# Autodesk Inventor assembly: Bracket Assembly MK6
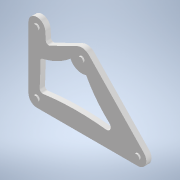
[picture p0: Inventor's stored thumbnail of the model, 180x180]
Saved by Autodesk Inventor 2021 (Build 250183000, 183)
## iProperties
Created: 2021-05-12
Part Number: Bracket Assembly MK6
Document SubType Name: Assembly
Designer: Jawal
Author: Jawal
## Documents named in this file (3)
- C:\Users\Jawal\Documents\UNI\PART III\Semester 1\MECHENG 334\Project B\Concept Design\Bracket Assembly MK6.iam
- C:\Users\Jawal\Documents\UNI\PART III\Semester 1\MECHENG 334\Project B\Concept Design\Pin.ipt
- C:\Users\Jawal\Documents\UNI\PART III\Semester 1\MECHENG 334\Project B\Concept Design\Bracket Concept MK6.ipt
## Components (5 placed, 2 different names)
1. Pin:1 — Rigid:1
2. Pin:2 — Rigid:3
3. Pin:3 — Rigid:4
4. Pin:4 — Rigid:2
5. Bracket Concept MK6:1 — Rigid:1, Rigid:2, Rigid:3, Rigid:4
## Relationships (4: WeldJoint 4)
- Rigid:1 [WeldJoint]: Pin:1 ↔ Bracket Concept MK6:1
- Rigid:2 [WeldJoint]: Pin:4 ↔ Bracket Concept MK6:1
- Rigid:3 [WeldJoint]: Pin:2 ↔ Bracket Concept MK6:1
- Rigid:4 [WeldJoint]: Pin:3 ↔ Bracket Concept MK6:1
